# Autodesk Inventor assembly: Test
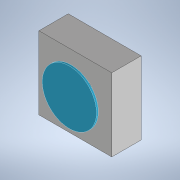
[picture p0: Inventor's stored thumbnail of the model, 180x180]
Saved by Autodesk Inventor 2022 (Build 260153000, 153)
## iProperties
Created: 2022-02-27
Part Number: Test
Document SubType Name: Assembly
Designer: alexo
Author: alexo
## Documents named in this file (4)
- C:\Users\alexo\Documents\Inventor\Scanner3D\Test.iam
- C:\Users\alexo\Documents\Inventor\Scanner3D\Base.ipt
- C:\Users\alexo\Documents\Inventor\Scanner3D\StepperMotor.ipt
- C:\Users\alexo\Documents\Inventor\Scanner3D\infoeducatia 2022\proiectare\pat_scanare\pat.iam
## Components (4 placed, 3 different names)
1. Base:1 — Mate:1, Mate:2, Mate:3, Mate:4, Rigid:1
2. StepperMotor:1 — Mate:1, Mate:2, Mate:3
3. StepperMotor:2 — Mate:4
4. pat:1 [sub-assembly] — Rigid:1
## Relationships (5: Mate 4, WeldJoint 1)
- Mate:1: Base:1 ↔ StepperMotor:1
- Mate:2: Base:1 ↔ StepperMotor:1
- Mate:3: Base:1 ↔ StepperMotor:1
- Mate:4: Base:1 ↔ StepperMotor:2
- Rigid:1 [WeldJoint] (-1 mm): Base:1 ↔ pat:1
